# Autodesk Inventor assembly: 組合
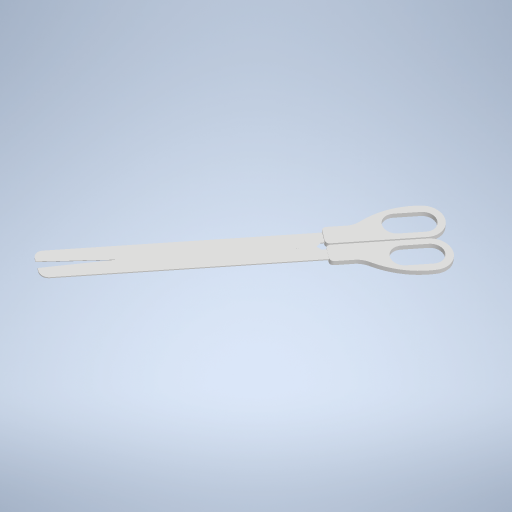
[picture p0: Inventor's stored thumbnail of the model, 512x512]
Saved by Autodesk Inventor 2024.2 (Build 282272000, 272)
## iProperties
Created: 2024-05-16
Part Number: 組合
Document SubType Name: Assembly
Designer: User
Author: User
## Documents named in this file (4)
- C:\Users\User\OneDrive - 國立中山大學\桌面\創客基礎\0516\組合.iam
- C:\Users\User\OneDrive - 國立中山大學\桌面\創客基礎\0516\剪刀握柄.ipt
- C:\Users\User\OneDrive - 國立中山大學\桌面\創客基礎\0516\刀柄.ipt
- C:\Users\User\OneDrive - 國立中山大學\桌面\創客基礎\0516\圓柱.ipt
## Components (5 placed, 3 different names)
1. 刀柄:1 — 貼合:1, 貼合:2, 齊平:1, 齊平:2, 貼合:4, 貼合:5, 貼合:8
2. 刀柄:2 — 貼合:1, 貼合:2, 貼合:3, 齊平:2, 貼合:6, 貼合:7, 貼合:9
3. 圓柱:1 — 貼合:3, 齊平:1
4. 剪刀握柄:1 — 貼合:4, 貼合:5, 貼合:8
5. 剪刀握柄:2 — 貼合:6, 貼合:7, 貼合:9
## Relationships (11: Mate 9, Flush 2)
- 貼合:1 [Mate]: 刀柄:1 ↔ 刀柄:2
- 貼合:2 [Mate]: 刀柄:1 ↔ 刀柄:2
- 貼合:3 [Mate]: 刀柄:2 ↔ 圓柱:1
- 齊平:1 [Flush] (-0.25 mm): 刀柄:1 ↔ 圓柱:1
- 齊平:2 [Flush]: 刀柄:1 ↔ 刀柄:2
- 貼合:4 [Mate]: 刀柄:1 ↔ 剪刀握柄:1
- 貼合:5 [Mate]: 刀柄:1 ↔ 剪刀握柄:1
- 貼合:6 [Mate]: 刀柄:2 ↔ 剪刀握柄:2
- 貼合:7 [Mate]: 刀柄:2 ↔ 剪刀握柄:2
- 貼合:8 [Mate]: 刀柄:1 ↔ 剪刀握柄:1
- 貼合:9 [Mate]: 刀柄:2 ↔ 剪刀握柄:2
